# Autodesk Inventor assembly: !Drivebay Left
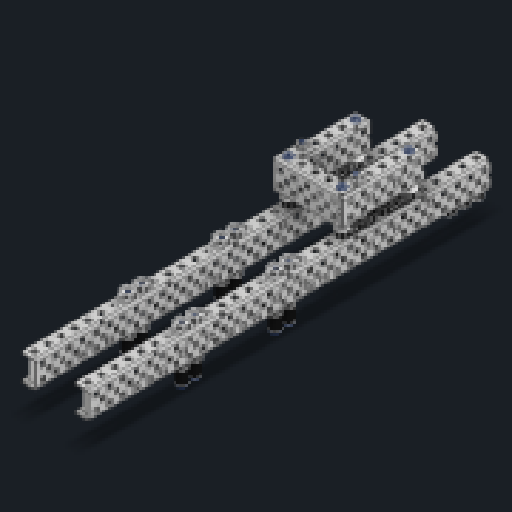
[picture p0: Inventor's stored thumbnail of the model, 512x512]
Saved by Autodesk Inventor 2025.1 (Build 291241000, 241)
## iProperties
Created: 2024-11-04
Part Number: !Drivebay Left
Document SubType Name: Assembly
Designer: avere
Author: avere
## Documents named in this file (4)
- C:\Users\avere\VEX\High Stakes\CAD\V3\Chassis\Drivebay Left\Structure.iam
- C:\Users\avere\VEX\High Stakes\CAD\V3\Chassis\Drivebay Left\Outer Channel.iam
- C:\Users\avere\VEX\High Stakes\CAD\V3\Chassis\Drivebay Left\Inner Channel.iam
- C:\Users\avere\VEX\High Stakes\CAD\V3\Chassis\Drivebay Left\Custom Parts\Knotched Alu C 2x2x2x5.ipt
## Components (3 placed, 3 different names)
1. Outer Channel:1 [sub-assembly] — Mate:1, Mate:2, Mate:3, Insert:1
2. Inner Channel:1 [sub-assembly] — Mate:1, Mate:2, Mate:3, Mate:4
3. Knotched Alu C 2x2x2x5:1 — Insert:1, Mate:4
## Relationships (5: Mate 4, Insert 1)
- Mate:1 (50.8 mm): Outer Channel:1 ↔ Inner Channel:1
- Mate:2: Outer Channel:1 ↔ Inner Channel:1
- Mate:3: Outer Channel:1 ↔ Inner Channel:1
- Insert:1: Outer Channel:1 ↔ Knotched Alu C 2x2x2x5:1
- Mate:4: Inner Channel:1 ↔ Knotched Alu C 2x2x2x5:1
